# Autodesk Inventor assembly: CanSat
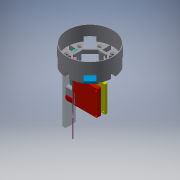
[picture p0: Inventor's stored thumbnail of the model, 180x180]
Saved by Autodesk Inventor 2018 (Build 220112000, 112)
## iProperties
Created: 2018-05-01
Part Number: CanSat
Document SubType Name: Assembly
Designer: suchanek
Author: suchanek
## Documents named in this file (13)
- C:\Users\sucha\programming\CanSat\CanSat2.0\Schematics\Model\CanSat.iam
- C:\Users\sucha\programming\CanSat\CanSat2.0\Schematics\Model\Hull_middle.ipt
- C:\Users\sucha\programming\CanSat\CanSat2.0\Schematics\Model\Hull_batt_pillar.ipt
- C:\Users\sucha\programming\CanSat\CanSat2.0\Schematics\Model\Circuit.ipt
- C:\Users\sucha\programming\CanSat\CanSat2.0\Schematics\Model\Motor_drivers.ipt
- C:\Users\sucha\programming\CanSat\CanSat2.0\Schematics\Model\Hull_main.ipt
- C:\Users\sucha\programming\CanSat\CanSat2.0\Schematics\Model\Circuit_center.ipt
- C:\Users\sucha\programming\CanSat\CanSat2.0\Schematics\Model\Arm.ipt
- C:\Users\sucha\programming\CanSat\CanSat2.0\Schematics\Model\Motor_holder.ipt
- C:\Users\sucha\programming\CanSat\CanSat2.0\Schematics\Model\Motor.ipt
- C:\Users\sucha\programming\CanSat\CanSat2.0\Schematics\Model\Rotor.ipt
- C:\Users\sucha\programming\CanSat\CanSat2.0\Schematics\Model\Flight_controler.ipt
- C:\Users\sucha\programming\CanSat\CanSat2.0\Schematics\Model\SIM808.ipt
## Components (15 placed, 12 different names)
1. Hull_middle:1 — Rotational:2, Angle:2, Rotational:3, Flush:2, Angle:5, Angle:6, Angle:7
2. Circuit:1 — Rotational:2, Angle:2, Angle:3
3. Motor_drivers:1 — Flush:1, Angle:4, Cylindrical:1, Mate:1
4. Hull_main:1 — Rotational:1, Angle:1, Rotational:3, Angle:3, Flush:1, Angle:4, Cylindrical:1, Rotational:4, Mate:3
5. Circuit_center:1 — Planar:1, Flush:2
6. Arm:1 — Rotational:4, Rigid:1
7. Motor_holder:1 — Rigid:1, Rigid:2
8. Motor:1 — Rigid:2, Rotational:5
9. Rotor:1 — Rotational:5
10. Flight_controler:1 — Mate:1, Angle:5, Flush:3, Mate:2, Symmetry:1, Symmetry:2, Flush:4
11. SIM808:1 — Flush:3, Mate:2, Symmetry:1, Symmetry:2, Flush:4
12. Hull_batt_pillar:1 — Rotational:1, Angle:1
13. Hull_batt_pillar:2 — Planar:1
14. Hull_batt_pillar:3
15. Hull_batt_pillar:4
## Component patterns: (4 elements, first: Hull_batt_pillar:1)
## Relationships (27: Angle 7, RevoluteJoint 5, Mate 5, Flush 4, WeldJoint 2, Symmetry 2, CylindricalJoint 1, PlanarJoint 1)
- Rotational:1 [RevoluteJoint]: Hull_main:1 ↔ Hull_batt_pillar:1
- Angle:1 (0 deg): Hull_main:1 ↔ Hull_batt_pillar:1
- Rotational:2 [RevoluteJoint]: Hull_middle:1 ↔ Circuit:1
- Angle:2 (0 deg): Hull_middle:1 ↔ Circuit:1
- Rotational:3 [RevoluteJoint]: Hull_middle:1 ↔ Hull_main:1
- Angle:3 (0 deg): Circuit:1 ↔ Hull_main:1
- Flush:1 (12 mm): Motor_drivers:1 ↔ Hull_main:1
- Angle:4 (0 deg): Motor_drivers:1 ↔ Hull_main:1
- Cylindrical:1: Motor_drivers:1 ↔ Hull_main:1
- Planar:1 (0.5 mm): Circuit_center:1 ↔ Hull_batt_pillar:2
- Flush:2 (3 mm): Hull_middle:1 ↔ Circuit_center:1
- Rotational:4 [RevoluteJoint] (-0.15 mm): Hull_main:1 ↔ Arm:1
- Rigid:1 [WeldJoint]: Arm:1 ↔ Motor_holder:1
- Rigid:2 [WeldJoint]: Motor_holder:1 ↔ Motor:1
- Rotational:5 [RevoluteJoint]: Motor:1 ↔ Rotor:1
- Mate:1 (5 mm): Motor_drivers:1 ↔ Flight_controler:1
- Angle:5 (0 deg): Hull_middle:1 ↔ Flight_controler:1
- Flush:3: Flight_controler:1 ↔ SIM808:1
- Mate:2 (5 mm): Flight_controler:1 ↔ SIM808:1
- Mate:3: Hull_main:1
- Mate:4
- Angle:6 (90 deg): Hull_middle:1
- Mate:5
- Angle:7 (90 deg): Hull_middle:1
- Symmetry:1: Flight_controler:1 ↔ SIM808:1
- Symmetry:2: Flight_controler:1 ↔ SIM808:1
- Flush:4 (-0.5 mm): Flight_controler:1 ↔ SIM808:1
